# Autodesk Inventor assembly: Prueba3_V2
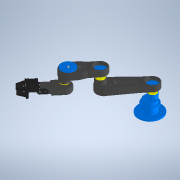
[picture p0: Inventor's stored thumbnail of the model, 180x180]
Saved by Autodesk Inventor 2021 (Build 250183000, 183)
## iProperties
Created: 2022-04-22
Part Number: Prueba3_V2
Document SubType Name: Assembly
Designer: Alcatraz
Author: Alcatraz
## Documents named in this file (5)
- F:\Tesis\TESIS\Matlab\Pruebas\Prueba3_Simulacion2\Prueba3_V2.iam
- F:\Tesis\TESIS\Matlab\Pruebas\Prueba3_Simulacion2\Eslabon1.ipt
- F:\Tesis\TESIS\Matlab\Pruebas\Prueba3_Simulacion2\Eslabon2.ipt
- F:\Tesis\TESIS\Matlab\Pruebas\Prueba3_Simulacion2\Eslabon3.ipt
- F:\Tesis\TESIS\Matlab\Pruebas\Prueba3_Simulacion2\Base.ipt
## Components (4 placed, 4 different names)
1. Eslabon1:1 — De rotación:2, De rotación:4
2. Eslabon2:1 — De rotación:2, De rotación:3
3. Eslabon3:1 — De rotación:3
4. Base:1 — De rotación:4
## Relationships (3: RevoluteJoint 3)
- De rotación:2 [RevoluteJoint]: Eslabon1:1 ↔ Eslabon2:1
- De rotación:3 [RevoluteJoint]: Eslabon2:1 ↔ Eslabon3:1
- De rotación:4 [RevoluteJoint]: Eslabon1:1 ↔ Base:1
